# Autodesk Inventor assembly: NASA-20
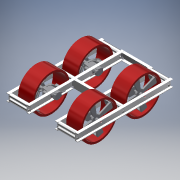
[picture p0: Inventor's stored thumbnail of the model, 180x180]
Saved by Autodesk Inventor 2019 (Build 230136000, 136)
## iProperties
Created: 2019-09-05
Part Number: NASA-20
Document SubType Name: Assembly
Designer: Rick Szalay
RuleStatus: InUse
Author: Rick Szalay
## Documents named in this file (10)
- C:\Users\Rick Szalay\Documents\Inventor\NASA 20\NASA-20\NASA-20.iam
- C:\Users\Rick Szalay\Documents\Inventor\NASA 20\NASA-20\A428.ipt
- C:\Users\Rick Szalay\Documents\Inventor\NASA 20\NASA-20\NASA-20-WH-01.ipt
- C:\Users\Rick Szalay\Documents\Inventor\NASA 20\NASA-20\NASA-20-WT-01.ipt
- C:\Users\Rick Szalay\Documents\Inventor\NASA 20\NASA-20\FR\NASA-20-FR.iam
- C:\Users\Rick Szalay\Documents\Inventor\NASA 20\NASA-20\FR\NASA-20-TB-01.ipt
- C:\Users\Rick Szalay\Documents\Inventor\NASA 20\NASA-20\FR\NASA-20-OP-01.ipt
- C:\Users\Rick Szalay\Documents\Inventor\NASA 20\NASA-20\FR\NASA-20-MP-01.ipt
- C:\Users\Rick Szalay\Documents\Inventor\Content Center Files\R2019\en-US\ANSI B18.2.1(3)\ANSI B18.2.1 - 1_4-20 UNC - 5.5(3).ipt
- C:\Users\Rick Szalay\Documents\Inventor\Content Center Files\R2019\en-US\ANSI B18.2.2(09)\ANSI B18.2.2 - 1_4 - 20(2).ipt
## Components (55 placed, 9 different names)
1. A428:1 — Mate:38, Mate:39, Flush:28, Mate:41
2. NASA-20-WH-01:1 — Mate:6, Flush:9, Mate:40, Mate:41
3. NASA-20-WT-01:1 — Mate:6, Flush:9, Mate:61, Tangent:1
4. NASA-20-FR:1 [sub-assembly] — Mate:20, Mate:21, Flush:13, Mate:22, Mate:23, Mate:24, Mate:25, Mate:26, Mate:27, Mate:28, Mate:29, Mate:30, Mate:31, Mate:32, Mate:33, Mate:34, Mate:35, Flush:26, Flush:27, Flush:29, Mate:42, Mate:58, Flush:36, Mate:59, Mate:60, Flush:37, Flush:38, Insert:13, Insert:14, Insert:15, Insert:16, Insert:17, Insert:18, Insert:19, Insert:20, Insert:21, Insert:22, Insert:23, Insert:24
5. NASA-20-TB-01:1 — Flush:14, Mate:22, Mate:23
6. NASA-20-TB-01:2 — Flush:14, Flush:15, Mate:24, Mate:36
7. NASA-20-TB-01:3 — Flush:15, Flush:16, Mate:25
8. NASA-20-TB-01:4 — Flush:16, Flush:17, Mate:26
9. NASA-20-TB-01:5 — Flush:17, Flush:18, Mate:27
10. NASA-20-TB-01:6 — Flush:18, Mate:28
11. NASA-20-TB-01:7 — Mate:34, Mate:37
12. NASA-20-TB-01:8 — Mate:35
13. NASA-20-TB-01:9 — Mate:30
14. NASA-20-TB-01:10 — Mate:33
15. NASA-20-TB-01:11 — Mate:32
16. NASA-20-TB-01:12 — Mate:29, Mate:31
17. NASA-20-OP-01:1 — Flush:24, Flush:25, Mate:37, Flush:26, Flush:27, Mate:63, Insert:7, Insert:8, Insert:9, Insert:10, Insert:11, Insert:12
18. NASA-20-OP-01:2 — Flush:24, Flush:25, Mate:36, Insert:1, Insert:2, Insert:3, Insert:4, Insert:5, Insert:6
19. NASA-20-MP-01:1 — Mate:38, Mate:39, Flush:28, Mate:40, Flush:29, Mate:42
20. A428:2
21. NASA-20-WH-01:2
22. NASA-20-WT-01:2 — Mate:62, Tangent:1
23. NASA-20-MP-01:2 — Mate:58, Flush:36
24. A428:3
25. NASA-20-WH-01:3
26. NASA-20-WT-01:3 — Mate:62, Mate:63
27. NASA-20-MP-01:3 — Mate:59, Flush:37
28. A428:4
29. NASA-20-WH-01:4
30. NASA-20-WT-01:4 — Mate:61
31. NASA-20-MP-01:4 — Mate:60, Flush:38
32. Hex Cap Screw - Inch 1/4-20 UNC - 5.5:1 — Insert:1
33. Hex Cap Screw - Inch 1/4-20 UNC - 5.5:2 — Insert:2
34. Hex Cap Screw - Inch 1/4-20 UNC - 5.5:3 — Insert:3
35. Hex Cap Screw - Inch 1/4-20 UNC - 5.5:4 — Insert:4
36. Hex Cap Screw - Inch 1/4-20 UNC - 5.5:5 — Insert:5
37. Hex Cap Screw - Inch 1/4-20 UNC - 5.5:6 — Insert:6
38. Hex Cap Screw - Inch 1/4-20 UNC - 5.5:7 — Insert:7
39. Hex Cap Screw - Inch 1/4-20 UNC - 5.5:8 — Insert:8
40. Hex Cap Screw - Inch 1/4-20 UNC - 5.5:9 — Insert:9
41. Hex Cap Screw - Inch 1/4-20 UNC - 5.5:10 — Insert:10
42. Hex Cap Screw - Inch 1/4-20 UNC - 5.5:11 — Insert:11
43. Hex Cap Screw - Inch 1/4-20 UNC - 5.5:12 — Insert:12
44. Hex Nut - Inch 1/4 - 20:1 — Insert:13
45. Hex Nut - Inch 1/4 - 20:2 — Insert:14
46. Hex Nut - Inch 1/4 - 20:3 — Insert:15
47. Hex Nut - Inch 1/4 - 20:4 — Insert:16
48. Hex Nut - Inch 1/4 - 20:5 — Insert:17
49. Hex Nut - Inch 1/4 - 20:6 — Insert:18
50. Hex Nut - Inch 1/4 - 20:7 — Insert:19
51. Hex Nut - Inch 1/4 - 20:8 — Insert:20
52. Hex Nut - Inch 1/4 - 20:9 — Insert:21
53. Hex Nut - Inch 1/4 - 20:10 — Insert:22
54. Hex Nut - Inch 1/4 - 20:11 — Insert:23
55. Hex Nut - Inch 1/4 - 20:12 — Insert:24
## Relationships (97: Mate 45, Flush 27, Insert 24, Tangent 1)
- Mate:6: NASA-20-WH-01:1 ↔ NASA-20-WT-01:1
- Flush:9 (19.05 mm): NASA-20-WH-01:1 ↔ NASA-20-WT-01:1
- Mate:20: NASA-20-FR:1
- Mate:21: NASA-20-FR:1
- Flush:13: NASA-20-FR:1
- Flush:14: NASA-20-TB-01:1 ↔ NASA-20-TB-01:2
- Flush:15: NASA-20-TB-01:2 ↔ NASA-20-TB-01:3
- Flush:16: NASA-20-TB-01:3 ↔ NASA-20-TB-01:4
- Flush:17: NASA-20-TB-01:4 ↔ NASA-20-TB-01:5
- Flush:18: NASA-20-TB-01:5 ↔ NASA-20-TB-01:6
- Mate:22: NASA-20-FR:1 ↔ NASA-20-TB-01:1
- Mate:23: NASA-20-FR:1 ↔ NASA-20-TB-01:1
- Mate:24: NASA-20-FR:1 ↔ NASA-20-TB-01:2
- Mate:25: NASA-20-FR:1 ↔ NASA-20-TB-01:3
- Mate:26: NASA-20-FR:1 ↔ NASA-20-TB-01:4
- Mate:27: NASA-20-FR:1 ↔ NASA-20-TB-01:5
- Mate:28: NASA-20-FR:1 ↔ NASA-20-TB-01:6
- [Flush]: NASA-20-TB-01:7 ↔ NASA-20-TB-01:8
- [Flush]: NASA-20-TB-01:8 ↔ NASA-20-TB-01:9
- [Flush]: NASA-20-TB-01:9 ↔ NASA-20-TB-01:10
- [Flush]: NASA-20-TB-01:10 ↔ NASA-20-TB-01:11
- [Flush]: NASA-20-TB-01:11 ↔ NASA-20-TB-01:12
- Mate:29: NASA-20-FR:1 ↔ NASA-20-TB-01:12
- Mate:30: NASA-20-FR:1 ↔ NASA-20-TB-01:9
- Mate:31: NASA-20-FR:1 ↔ NASA-20-TB-01:12
- Mate:32: NASA-20-FR:1 ↔ NASA-20-TB-01:11
- Mate:33: NASA-20-FR:1 ↔ NASA-20-TB-01:10
- Mate:34: NASA-20-FR:1 ↔ NASA-20-TB-01:7
- Mate:35: NASA-20-FR:1 ↔ NASA-20-TB-01:8
- Flush:24: NASA-20-OP-01:1 ↔ NASA-20-OP-01:2
- Flush:25: NASA-20-OP-01:1 ↔ NASA-20-OP-01:2
- Mate:36: NASA-20-TB-01:2 ↔ NASA-20-OP-01:2
- Mate:37: NASA-20-TB-01:7 ↔ NASA-20-OP-01:1
- Flush:26: NASA-20-FR:1 ↔ NASA-20-OP-01:1
- Flush:27: NASA-20-FR:1 ↔ NASA-20-OP-01:1
- Mate:38: A428:1 ↔ NASA-20-MP-01:1
- Mate:39: A428:1 ↔ NASA-20-MP-01:1
- Flush:28: A428:1 ↔ NASA-20-MP-01:1
- Mate:40 (1.5875 mm): NASA-20-WH-01:1 ↔ NASA-20-MP-01:1
- Mate:41: A428:1 ↔ NASA-20-WH-01:1
- Flush:29: NASA-20-FR:1 ↔ NASA-20-MP-01:1
- Mate:42: NASA-20-FR:1 ↔ NASA-20-MP-01:1
- [Mate]: NASA-20-WH-01:2 ↔ NASA-20-WT-01:2
- [Flush] (19.05 mm): NASA-20-WH-01:2 ↔ NASA-20-WT-01:2
- [Mate]: A428:2 ↔ NASA-20-MP-01:2
- [Mate]: A428:2 ↔ NASA-20-MP-01:2
- [Flush]: A428:2 ↔ NASA-20-MP-01:2
- [Mate] (1.5875 mm): NASA-20-WH-01:2 ↔ NASA-20-MP-01:2
- [Mate]: A428:2 ↔ NASA-20-WH-01:2
- [Mate]: NASA-20-WH-01:3 ↔ NASA-20-WT-01:3
- [Flush] (19.05 mm): NASA-20-WH-01:3 ↔ NASA-20-WT-01:3
- [Mate]: A428:3 ↔ NASA-20-MP-01:3
- [Mate]: A428:3 ↔ NASA-20-MP-01:3
- [Flush]: A428:3 ↔ NASA-20-MP-01:3
- [Mate] (1.5875 mm): NASA-20-WH-01:3 ↔ NASA-20-MP-01:3
- [Mate]: A428:3 ↔ NASA-20-WH-01:3
- [Mate]: NASA-20-WH-01:4 ↔ NASA-20-WT-01:4
- [Flush] (19.05 mm): NASA-20-WH-01:4 ↔ NASA-20-WT-01:4
- [Mate]: A428:4 ↔ NASA-20-MP-01:4
- [Mate]: A428:4 ↔ NASA-20-MP-01:4
- [Flush]: A428:4 ↔ NASA-20-MP-01:4
- [Mate] (1.5875 mm): NASA-20-WH-01:4 ↔ NASA-20-MP-01:4
- [Mate]: A428:4 ↔ NASA-20-WH-01:4
- Mate:58: NASA-20-FR:1 ↔ NASA-20-MP-01:2
- Flush:36: NASA-20-FR:1 ↔ NASA-20-MP-01:2
- Mate:59: NASA-20-FR:1 ↔ NASA-20-MP-01:3
- Mate:60: NASA-20-FR:1 ↔ NASA-20-MP-01:4
- Flush:37: NASA-20-FR:1 ↔ NASA-20-MP-01:3
- Flush:38: NASA-20-FR:1 ↔ NASA-20-MP-01:4
- Mate:61: NASA-20-WT-01:1 ↔ NASA-20-WT-01:4
- Mate:62: NASA-20-WT-01:2 ↔ NASA-20-WT-01:3
- Tangent:1 (50.8 mm): NASA-20-WT-01:1 ↔ NASA-20-WT-01:2
- Mate:63: NASA-20-OP-01:1 ↔ NASA-20-WT-01:3
- Insert:1 (-139.065 mm): NASA-20-OP-01:2 ↔ Hex Cap Screw - Inch 1/4-20 UNC - 5.5:1
- Insert:2 (-139.065 mm): NASA-20-OP-01:2 ↔ Hex Cap Screw - Inch 1/4-20 UNC - 5.5:2
- Insert:3 (-139.065 mm): NASA-20-OP-01:2 ↔ Hex Cap Screw - Inch 1/4-20 UNC - 5.5:3
- Insert:4 (-139.065 mm): NASA-20-OP-01:2 ↔ Hex Cap Screw - Inch 1/4-20 UNC - 5.5:4
- Insert:5 (-139.065 mm): NASA-20-OP-01:2 ↔ Hex Cap Screw - Inch 1/4-20 UNC - 5.5:5
- Insert:6 (-139.065 mm): NASA-20-OP-01:2 ↔ Hex Cap Screw - Inch 1/4-20 UNC - 5.5:6
- Insert:7 (-139.065 mm): NASA-20-OP-01:1 ↔ Hex Cap Screw - Inch 1/4-20 UNC - 5.5:7
- Insert:8 (-139.065 mm): NASA-20-OP-01:1 ↔ Hex Cap Screw - Inch 1/4-20 UNC - 5.5:8
- Insert:9 (-139.065 mm): NASA-20-OP-01:1 ↔ Hex Cap Screw - Inch 1/4-20 UNC - 5.5:9
- Insert:10 (-139.065 mm): NASA-20-OP-01:1 ↔ Hex Cap Screw - Inch 1/4-20 UNC - 5.5:10
- Insert:11 (-139.065 mm): NASA-20-OP-01:1 ↔ Hex Cap Screw - Inch 1/4-20 UNC - 5.5:11
- Insert:12 (-139.065 mm): NASA-20-OP-01:1 ↔ Hex Cap Screw - Inch 1/4-20 UNC - 5.5:12
- Insert:13: NASA-20-FR:1 ↔ Hex Nut - Inch 1/4 - 20:1
- Insert:14: NASA-20-FR:1 ↔ Hex Nut - Inch 1/4 - 20:2
- Insert:15: NASA-20-FR:1 ↔ Hex Nut - Inch 1/4 - 20:3
- Insert:16: NASA-20-FR:1 ↔ Hex Nut - Inch 1/4 - 20:4
- Insert:17: NASA-20-FR:1 ↔ Hex Nut - Inch 1/4 - 20:5
- Insert:18: NASA-20-FR:1 ↔ Hex Nut - Inch 1/4 - 20:6
- Insert:19: NASA-20-FR:1 ↔ Hex Nut - Inch 1/4 - 20:7
- Insert:20: NASA-20-FR:1 ↔ Hex Nut - Inch 1/4 - 20:8
- Insert:21: NASA-20-FR:1 ↔ Hex Nut - Inch 1/4 - 20:9
- Insert:22: NASA-20-FR:1 ↔ Hex Nut - Inch 1/4 - 20:10
- Insert:23: NASA-20-FR:1 ↔ Hex Nut - Inch 1/4 - 20:11
- Insert:24: NASA-20-FR:1 ↔ Hex Nut - Inch 1/4 - 20:12
## Named parameters: d53_d41 = 0 mm, d54_d42 = 0 mm, d55_d43 = 0 mm, d56_d44 = 0 mm, d57_d45 = 0 mm, d78_d71 = 0 mm, d79_d72 = 0 mm, d80_d73 = 0 mm, d81_d74 = 1.5875 mm, d82_d75 = 0 mm, d83_d14 = 0 mm, d84_d15 = 19.05 mm, d85_d71 = 0 mm, d86_d72 = 0 mm, d87_d73 = 0 mm, d88_d74 = 1.5875 mm, d89_d75 = 0 mm, d90_d14 = 0 mm, d91_d15 = 19.05 mm, d92_d71 = 0 mm, d93_d72 = 0 mm, d94_d73 = 0 mm, d95_d74 = 1.5875 mm, d96_d75 = 0 mm, d97_d14 = 0 mm, d98_d15 = 19.05 mm
